# Autodesk Inventor assembly: Durometer_Lead_Screw_Fixture
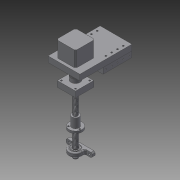
[picture p0: Inventor's stored thumbnail of the model, 180x180]
Saved by Autodesk Inventor 2015 (Build 190159000, 159)
## iProperties
Created: 2014-12-21
Part Number: Durometer_Lead_Screw_Fixture
Document SubType Name: Assembly
Designer: Drew
Author: Drew
## Documents named in this file (10)
- C:\Users\Drew\Dropbox\Durometer\Durometer_Assembly\Durometer_Lead_Screw_Fixture.iam
- C:\Users\Drew\Dropbox\Durometer\Durometer_Assembly\Lead_Screw_Fixture_Base.ipt
- C:\Users\Drew\Dropbox\Durometer\Durometer_Assembly\Stepper_Motor.ipt
- C:\Users\Drew\Dropbox\Durometer\Durometer_Assembly\Lead_Screw_Fixture_Side_Wall.ipt
- C:\Users\Drew\Dropbox\Durometer\Durometer_Assembly\Shaft_Coupler_5mm_10mm.ipt
- C:\Users\Drew\Dropbox\Durometer\Durometer_Assembly\Ball_Bearing_8600N140.ipt
- C:\Users\Drew\Dropbox\Durometer\Durometer_Assembly\Lead_Screw_Flange_Nut.ipt
- C:\Users\Drew\Dropbox\Durometer\Durometer_Assembly\Lead_Screw_10x2.ipt
- C:\Users\Drew\Dropbox\Durometer\Durometer_Assembly\Flange_Bearing_5448T5.ipt
- C:\Users\Drew\Dropbox\Durometer\Durometer_Assembly\Lead_Screw_Thrust_Bearing_Mount.ipt
## Components (10 placed, 9 different names)
1. Lead_Screw_Fixture_Base:1 — Mate:1, Mate:3, Mate:4, Mate:5, Mate:6, Mate:7, Mate:8, Mate:9, Mate:10, Mate:12, Mate:18, Mate:19
2. Stepper_Motor:1 — Mate:1, Mate:3, Mate:4, Mate:11
3. Lead_Screw_Fixture_Side_Wall:1 — Mate:5, Mate:6, Mate:7
4. Lead_Screw_Fixture_Side_Wall:2 — Mate:8, Mate:9, Mate:10
5. Shaft_Coupler_5mm_10mm:1 — Mate:11, Mate:12, Mate:13, Mate:14, Mate:16
6. Ball_Bearing_8600N140:1 — Mate:21
7. Lead_Screw_Flange_Nut:1 — Mate:17
8. Lead_Screw_10x2:1 — Mate:13, Mate:14, Mate:15, Mate:17, Mate:21
9. Flange_Bearing_5448T5:1 — Mate:15, Mate:16, Mate:20
10. Lead_Screw_Thrust_Bearing_Mount:1 — Mate:18, Mate:19, Mate:20
## Relationships (20: Mate 20)
- Mate:1: Lead_Screw_Fixture_Base:1 ↔ Stepper_Motor:1
- Mate:3: Lead_Screw_Fixture_Base:1 ↔ Stepper_Motor:1
- Mate:4: Lead_Screw_Fixture_Base:1 ↔ Stepper_Motor:1
- Mate:5: Lead_Screw_Fixture_Base:1 ↔ Lead_Screw_Fixture_Side_Wall:1
- Mate:6: Lead_Screw_Fixture_Base:1 ↔ Lead_Screw_Fixture_Side_Wall:1
- Mate:7: Lead_Screw_Fixture_Base:1 ↔ Lead_Screw_Fixture_Side_Wall:1
- Mate:8: Lead_Screw_Fixture_Base:1 ↔ Lead_Screw_Fixture_Side_Wall:2
- Mate:9: Lead_Screw_Fixture_Base:1 ↔ Lead_Screw_Fixture_Side_Wall:2
- Mate:10: Lead_Screw_Fixture_Base:1 ↔ Lead_Screw_Fixture_Side_Wall:2
- Mate:11: Stepper_Motor:1 ↔ Shaft_Coupler_5mm_10mm:1
- Mate:12 (2.54 mm): Lead_Screw_Fixture_Base:1 ↔ Shaft_Coupler_5mm_10mm:1
- Mate:13: Shaft_Coupler_5mm_10mm:1 ↔ Lead_Screw_10x2:1
- Mate:14: Shaft_Coupler_5mm_10mm:1 ↔ Lead_Screw_10x2:1
- Mate:15: Lead_Screw_10x2:1 ↔ Flange_Bearing_5448T5:1
- Mate:16: Shaft_Coupler_5mm_10mm:1 ↔ Flange_Bearing_5448T5:1
- Mate:17: Lead_Screw_Flange_Nut:1 ↔ Lead_Screw_10x2:1
- Mate:18: Lead_Screw_Fixture_Base:1 ↔ Lead_Screw_Thrust_Bearing_Mount:1
- Mate:19: Lead_Screw_Fixture_Base:1 ↔ Lead_Screw_Thrust_Bearing_Mount:1
- Mate:20: Flange_Bearing_5448T5:1 ↔ Lead_Screw_Thrust_Bearing_Mount:1
- Mate:21: Ball_Bearing_8600N140:1 ↔ Lead_Screw_10x2:1
